# Autodesk Inventor assembly: 足裏_1_1
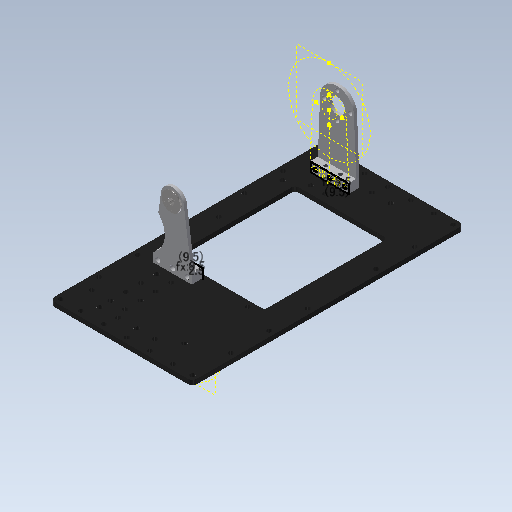
[picture p0: Inventor's stored thumbnail of the model, 512x512]
Saved by Autodesk Inventor 2020 (Build 240168000, 168)
## iProperties
Created: 2016-05-01
Part Number: 足裏_1_1
Document SubType Name: Assembly
Designer: hiroaki
Mass: 45.5975 g
Surface Area: 270.055 cm^2
Volume: 23.2522 cm^3
Density: 1.96099 g/cm^3
Author: hiroaki
## Documents named in this file (6)
- C:\Users\6343y\Documents\Inventor\GankenKun\OpenPlatform_ver3_0\下半身\足裏\足裏_1_1.iam
- C:\Users\6343y\Documents\Inventor\GankenKun\OpenPlatform_ver3_0\下半身\足裏\足裏_メインフレーム_1_1.ipt
- C:\Users\6343y\Documents\Inventor\GankenKun\OpenPlatform_ver3_0\下半身\足裏\足裏_メインフレーム_1_2.ipt
- C:\Users\6343y\Documents\Inventor\GankenKun\OpenPlatform_ver3_0\下半身\足裏\足裏_サブフレーム_1_1.ipt
- C:\Users\6343y\Documents\Inventor\GankenKun\OpenPlatform_ver3_0\既製品\NSK_RB_F694ZZ\F694ZZ.iam
- C:\Users\6343y\Documents\Inventor\GankenKun\OpenPlatform_ver3_0\下半身\足裏\足裏_メインフレーム_2_3.ipt
## Components (6 placed, 5 different names)
1. 足裏_メインフレーム_1_1:1 — メイト:1, フラッシュ:1, フラッシュ:2, メイト:2, フラッシュ:3, 挿入:4, 挿入:5, 挿入:6
2. 足裏_メインフレーム_1_2:1 — メイト:2, フラッシュ:3, 挿入:1, 挿入:2, 挿入:3, 挿入:12
3. 足裏_サブフレーム_1_1:1 — 挿入:1, 挿入:2, 挿入:3, 挿入:15, 挿入:16
4. 足裏_サブフレーム_1_1:2 — 挿入:4, 挿入:5, 挿入:6, 挿入:13, 挿入:14
5. F694ZZ:1 [sub-assembly] — 挿入:12
6. 足裏_メインフレーム_2_3:1 — 挿入:13, 挿入:14, 挿入:15, 挿入:16
## Relationships (16: Insert 11, Flush 3, Mate 2)
- メイト:1 [Mate]: 足裏_メインフレーム_1_1:1
- フラッシュ:1 [Flush]: 足裏_メインフレーム_1_1:1
- フラッシュ:2 [Flush] (50.5 mm): 足裏_メインフレーム_1_1:1
- メイト:2 [Mate]: 足裏_メインフレーム_1_1:1 ↔ 足裏_メインフレーム_1_2:1
- フラッシュ:3 [Flush]: 足裏_メインフレーム_1_1:1 ↔ 足裏_メインフレーム_1_2:1
- 挿入:1 [Insert]: 足裏_メインフレーム_1_2:1 ↔ 足裏_サブフレーム_1_1:1
- 挿入:2 [Insert]: 足裏_メインフレーム_1_2:1 ↔ 足裏_サブフレーム_1_1:1
- 挿入:3 [Insert]: 足裏_メインフレーム_1_2:1 ↔ 足裏_サブフレーム_1_1:1
- 挿入:4 [Insert]: 足裏_メインフレーム_1_1:1 ↔ 足裏_サブフレーム_1_1:2
- 挿入:5 [Insert]: 足裏_メインフレーム_1_1:1 ↔ 足裏_サブフレーム_1_1:2
- 挿入:6 [Insert]: 足裏_メインフレーム_1_1:1 ↔ 足裏_サブフレーム_1_1:2
- 挿入:12 [Insert]: 足裏_メインフレーム_1_2:1 ↔ F694ZZ:1
- 挿入:13 [Insert]: 足裏_サブフレーム_1_1:2 ↔ 足裏_メインフレーム_2_3:1
- 挿入:14 [Insert]: 足裏_サブフレーム_1_1:2 ↔ 足裏_メインフレーム_2_3:1
- 挿入:15 [Insert]: 足裏_サブフレーム_1_1:1 ↔ 足裏_メインフレーム_2_3:1
- 挿入:16 [Insert]: 足裏_サブフレーム_1_1:1 ↔ 足裏_メインフレーム_2_3:1
